# Autodesk Inventor assembly: ensambleInclinado
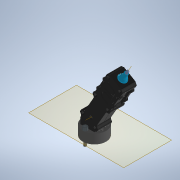
[picture p0: Inventor's stored thumbnail of the model, 180x180]
Saved by Autodesk Inventor 2021.5 (Build 255421000, 421)
## iProperties
Created: 2024-11-30
Part Number: ensambleInclinado
Document SubType Name: Assembly
Designer: Joho_
Mass: 153.406 g
Surface Area: 648.602 cm^2
Volume: 154.958 cm^3
Density: 0.989986 g/cm^3
Author: Joho_
## Documents named in this file (11)
- C:\Users\Joho_\Desktop\semestreN\robotica\laboratorios\lab01\CADs\ensambleInclinado.iam
- C:\Users\Joho_\Desktop\semestreN\robotica\laboratorios\lab01\CADs\baseSoporte.ipt
- C:\Users\Joho_\Desktop\semestreN\robotica\laboratorios\lab01\CADs\acopleInclinado30grados.ipt
- C:\Users\Joho_\Desktop\semestreN\robotica\laboratorios\lab01\CADs\marcador.ipt
- C:\Users\Joho_\Desktop\semestreN\robotica\laboratorios\lab01\CADs\tuercaM3.ipt
- C:\Users\Joho_\Desktop\semestreN\robotica\laboratorios\lab01\CADs\resortePlano1_2mmX3D.ipt
- C:\Users\Joho_\Desktop\semestreN\robotica\laboratorios\lab01\CADs\encajeTuerca.ipt
- C:\Users\Joho_\Desktop\semestreN\robotica\laboratorios\lab01\CADs\acopleInclinado30gradosReflejo.ipt
- C:\Users\Joho_\Desktop\semestreN\robotica\laboratorios\lab01\CADs\tonrilloM3x16mm.ipt
- C:\Users\Joho_\Desktop\semestreN\robotica\laboratorios\lab01\CADs\tonrilloM3x12mm.ipt
- C:\Users\Joho_\Desktop\semestreN\robotica\laboratorios\lab01\CADs\tornilloM6x30mm.ipt
## Components (25 placed, 10 different names)
1. baseSoporte:1 — Coincidencia:1, Coincidencia:2, Nivelación:1, Coincidencia:3, Coincidencia:4, Coincidencia:5, Coincidencia:35, Coincidencia:36, Coincidencia:37, Coincidencia:38
2. acopleInclinado30grados:1 — Coincidencia:3, Coincidencia:4, Coincidencia:5, Coincidencia:6, Nivelación:2, Ángulo:1, Coincidencia:8, Coincidencia:9, Coincidencia:10, Coincidencia:11, Coincidencia:12, Coincidencia:13, Ángulo:2, Ángulo:3, Coincidencia:14, Nivelación:6, Coincidencia:15, Coincidencia:16, Nivelación:8, Nivelación:9, Coincidencia:25, Coincidencia:26, Coincidencia:27, Coincidencia:28, Coincidencia:29, Coincidencia:30
3. marcador:1 — Coincidencia:6, Nivelación:2, Coincidencia:7
4. tuercaM3:1 — Nivelación:3, Coincidencia:8, Coincidencia:10, Ángulo:3, Coincidencia:33
5. tuercaM3:2 — Nivelación:3, Coincidencia:9, Ángulo:2, Coincidencia:32
6. resortePlano1_2mmX3D:1 — Coincidencia:11, Coincidencia:12, Coincidencia:13
7. encajeTuerca:1 — Nivelación:4, Nivelación:6, Nivelación:7, Coincidencia:15
8. encajeTuerca:2 — Nivelación:4, Coincidencia:14, Nivelación:7, Coincidencia:16
9. acopleInclinado30gradosReflejo:1 — Nivelación:8, Nivelación:9, Coincidencia:17, Coincidencia:18, Coincidencia:19, Coincidencia:20, Ángulo:4, Ángulo:5, Ángulo:6, Ángulo:7, Coincidencia:21, Coincidencia:22, Coincidencia:23, Coincidencia:24, Ángulo:8, Ángulo:9, Coincidencia:25
10. tuercaM3:3 — Nivelación:11, Coincidencia:17, Ángulo:7, Coincidencia:21
11. tuercaM3:4 — Nivelación:12, Coincidencia:20, Ángulo:6
12. tuercaM3:5 — Nivelación:10, Nivelación:12, Coincidencia:18, Ángulo:4
13. tuercaM3:6 — Nivelación:10, Nivelación:11, Coincidencia:19, Ángulo:5
14. tuercaM3:7 — Nivelación:13, Coincidencia:22, Coincidencia:24, Ángulo:9, Coincidencia:31
15. tuercaM3:8 — Nivelación:13, Coincidencia:23, Ángulo:8, Coincidencia:34
16. tonrilloM3x16mm:1 — Nivelación:14, Nivelación:15, Coincidencia:27
17. tonrilloM3x16mm:2 — Nivelación:14, Nivelación:16, Coincidencia:29, Coincidencia:30
18. tonrilloM3x16mm:3 — Nivelación:15, Coincidencia:26
19. tonrilloM3x16mm:4 — Nivelación:16, Coincidencia:28
20. tonrilloM3x12mm:1 — Nivelación:18, Nivelación:19, Coincidencia:32
21. tonrilloM3x12mm:2 — Nivelación:17, Nivelación:18, Coincidencia:31, Coincidencia:35
22. tonrilloM3x12mm:3 — Nivelación:19, Coincidencia:34
23. tonrilloM3x12mm:4 — Nivelación:17, Coincidencia:33
24. tornilloM6x30mm:1 — Nivelación:20, Coincidencia:36
25. tornilloM6x30mm:2 — Nivelación:20, Coincidencia:37, Coincidencia:38
## Relationships (66: Mate 38, Flush 19, Angle 9)
- Coincidencia:1 [Mate]: baseSoporte:1
- Coincidencia:2 [Mate]: baseSoporte:1
- Nivelación:1 [Flush]: baseSoporte:1
- Coincidencia:3 [Mate]: baseSoporte:1 ↔ acopleInclinado30grados:1
- Coincidencia:4 [Mate]: baseSoporte:1 ↔ acopleInclinado30grados:1
- Coincidencia:5 [Mate]: baseSoporte:1 ↔ acopleInclinado30grados:1
- Coincidencia:6 [Mate]: acopleInclinado30grados:1 ↔ marcador:1
- Nivelación:2 [Flush]: acopleInclinado30grados:1 ↔ marcador:1
- Coincidencia:7 [Mate]: marcador:1
- Ángulo:1 [Angle] (0 deg): acopleInclinado30grados:1
- Nivelación:3 [Flush]: tuercaM3:1 ↔ tuercaM3:2
- Coincidencia:8 [Mate]: acopleInclinado30grados:1 ↔ tuercaM3:1
- Coincidencia:9 [Mate]: acopleInclinado30grados:1 ↔ tuercaM3:2
- Coincidencia:10 [Mate]: acopleInclinado30grados:1 ↔ tuercaM3:1
- Coincidencia:11 [Mate]: acopleInclinado30grados:1 ↔ resortePlano1_2mmX3D:1
- Coincidencia:12 [Mate]: acopleInclinado30grados:1 ↔ resortePlano1_2mmX3D:1
- Coincidencia:13 [Mate]: acopleInclinado30grados:1 ↔ resortePlano1_2mmX3D:1
- Ángulo:2 [Angle] (0 deg): acopleInclinado30grados:1 ↔ tuercaM3:2
- Ángulo:3 [Angle] (0 deg): acopleInclinado30grados:1 ↔ tuercaM3:1
- Nivelación:4 [Flush]: encajeTuerca:1 ↔ encajeTuerca:2
- Coincidencia:14 [Mate]: acopleInclinado30grados:1 ↔ encajeTuerca:2
- Nivelación:6 [Flush]: acopleInclinado30grados:1 ↔ encajeTuerca:1
- Nivelación:7 [Flush]: encajeTuerca:1 ↔ encajeTuerca:2
- Coincidencia:15 [Mate]: acopleInclinado30grados:1 ↔ encajeTuerca:1
- Coincidencia:16 [Mate]: acopleInclinado30grados:1 ↔ encajeTuerca:2
- Nivelación:8 [Flush]: acopleInclinado30grados:1 ↔ acopleInclinado30gradosReflejo:1
- Nivelación:9 [Flush]: acopleInclinado30grados:1 ↔ acopleInclinado30gradosReflejo:1
- Nivelación:10 [Flush]: tuercaM3:5 ↔ tuercaM3:6
- Nivelación:11 [Flush]: tuercaM3:3 ↔ tuercaM3:6
- Nivelación:12 [Flush]: tuercaM3:4 ↔ tuercaM3:5
- Coincidencia:17 [Mate]: acopleInclinado30gradosReflejo:1 ↔ tuercaM3:3
- Coincidencia:18 [Mate]: acopleInclinado30gradosReflejo:1 ↔ tuercaM3:5
- Coincidencia:19 [Mate]: acopleInclinado30gradosReflejo:1 ↔ tuercaM3:6
- Coincidencia:20 [Mate]: acopleInclinado30gradosReflejo:1 ↔ tuercaM3:4
- Ángulo:4 [Angle] (0 deg): acopleInclinado30gradosReflejo:1 ↔ tuercaM3:5
- Ángulo:5 [Angle] (0 deg): acopleInclinado30gradosReflejo:1 ↔ tuercaM3:6
- Ángulo:6 [Angle] (0 deg): acopleInclinado30gradosReflejo:1 ↔ tuercaM3:4
- Ángulo:7 [Angle] (0 deg): acopleInclinado30gradosReflejo:1 ↔ tuercaM3:3
- Coincidencia:21 [Mate]: acopleInclinado30gradosReflejo:1 ↔ tuercaM3:3
- Nivelación:13 [Flush]: tuercaM3:7 ↔ tuercaM3:8
- Coincidencia:22 [Mate]: acopleInclinado30gradosReflejo:1 ↔ tuercaM3:7
- Coincidencia:23 [Mate]: acopleInclinado30gradosReflejo:1 ↔ tuercaM3:8
- Coincidencia:24 [Mate]: acopleInclinado30gradosReflejo:1 ↔ tuercaM3:7
- Ángulo:8 [Angle] (0 deg): acopleInclinado30gradosReflejo:1 ↔ tuercaM3:8
- Ángulo:9 [Angle] (0 deg): acopleInclinado30gradosReflejo:1 ↔ tuercaM3:7
- Coincidencia:25 [Mate]: acopleInclinado30grados:1 ↔ acopleInclinado30gradosReflejo:1
- Nivelación:14 [Flush]: tonrilloM3x16mm:1 ↔ tonrilloM3x16mm:2
- Nivelación:15 [Flush]: tonrilloM3x16mm:1 ↔ tonrilloM3x16mm:3
- Nivelación:16 [Flush]: tonrilloM3x16mm:2 ↔ tonrilloM3x16mm:4
- Coincidencia:26 [Mate]: acopleInclinado30grados:1 ↔ tonrilloM3x16mm:3
- Coincidencia:27 [Mate]: acopleInclinado30grados:1 ↔ tonrilloM3x16mm:1
- Coincidencia:28 [Mate]: acopleInclinado30grados:1 ↔ tonrilloM3x16mm:4
- Coincidencia:29 [Mate]: acopleInclinado30grados:1 ↔ tonrilloM3x16mm:2
- Coincidencia:30 [Mate]: acopleInclinado30grados:1 ↔ tonrilloM3x16mm:2
- Nivelación:17 [Flush]: tonrilloM3x12mm:2 ↔ tonrilloM3x12mm:4
- Nivelación:18 [Flush]: tonrilloM3x12mm:1 ↔ tonrilloM3x12mm:2
- Nivelación:19 [Flush]: tonrilloM3x12mm:1 ↔ tonrilloM3x12mm:3
- Coincidencia:31 [Mate]: tuercaM3:7 ↔ tonrilloM3x12mm:2
- Coincidencia:32 [Mate]: tuercaM3:2 ↔ tonrilloM3x12mm:1
- Coincidencia:33 [Mate]: tuercaM3:1 ↔ tonrilloM3x12mm:4
- Coincidencia:34 [Mate]: tuercaM3:8 ↔ tonrilloM3x12mm:3
- Coincidencia:35 [Mate]: baseSoporte:1 ↔ tonrilloM3x12mm:2
- Nivelación:20 [Flush]: tornilloM6x30mm:1 ↔ tornilloM6x30mm:2
- Coincidencia:36 [Mate]: baseSoporte:1 ↔ tornilloM6x30mm:1
- Coincidencia:37 [Mate]: baseSoporte:1 ↔ tornilloM6x30mm:2
- Coincidencia:38 [Mate]: baseSoporte:1 ↔ tornilloM6x30mm:2
